# Autodesk Inventor assembly: ElectronicsBatteryAssembly
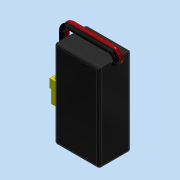
[picture p0: Inventor's stored thumbnail of the model, 180x180]
Saved by Autodesk Inventor 2017 (Build 210142000, 142)
## iProperties
Created: 2018-02-14
Part Number: ElectronicsBatteryAssembly
Document SubType Name: Assembly
Designer: Derek Wider
Author: Derek Wider
## Documents named in this file (3)
- G:\Projects\Submarine\Submarine-project\CAD\common\ElectronicsBatteryAssembly.iam
- G:\Projects\Submarine\Submarine-project\CAD\common\ElectronicsBatteryNoConnector.ipt
- G:\Projects\Submarine\Submarine-project\CAD\common\Connectors\XT60\XT60 Connector Female Connector.iam
## Components (2 placed, 2 different names)
1. ElectronicsBatteryNoConnector:1 — Mate:1, Mate:2, Angle:1
2. XT60 Connector Female Connector:1 [sub-assembly] — Mate:1, Mate:2, Angle:1
## Relationships (3: Mate 2, Angle 1)
- Mate:1: ElectronicsBatteryNoConnector:1 ↔ XT60 Connector Female Connector:1
- Mate:2: ElectronicsBatteryNoConnector:1 ↔ XT60 Connector Female Connector:1
- Angle:1 (0 deg): ElectronicsBatteryNoConnector:1 ↔ XT60 Connector Female Connector:1
